# Autodesk Inventor assembly: Anderson3x5
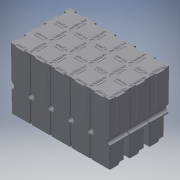
[picture p0: Inventor's stored thumbnail of the model, 180x180]
Saved by Autodesk Inventor 2018 (Build 220112000, 112)
## iProperties
Created: 2017-09-12
Part Number: Anderson3x5
Document SubType Name: Assembly
Designer: Srinity
Author: Srinity
## Documents named in this file (2)
- C:\Users\Srinity\Documents\DIY Projects\ModularFRCPlatform\Anderson3x5.iam
- C:\Users\Srinity\Documents\DIY Projects\ModularFRCPlatform\AndersonPP.ipt
## Components (15 placed, 1 different names)
1. AndersonPP:1
2. AndersonPP:2
3. AndersonPP:3
4. AndersonPP:4
5. AndersonPP:5
6. AndersonPP:6
7. AndersonPP:7
8. AndersonPP:8
9. AndersonPP:9
10. AndersonPP:10
11. AndersonPP:11
12. AndersonPP:12
13. AndersonPP:13
14. AndersonPP:14
15. AndersonPP:15
## Component patterns: (15 elements, first: AndersonPP:1)
